# Autodesk Inventor assembly: largeCapAssemblyGlued
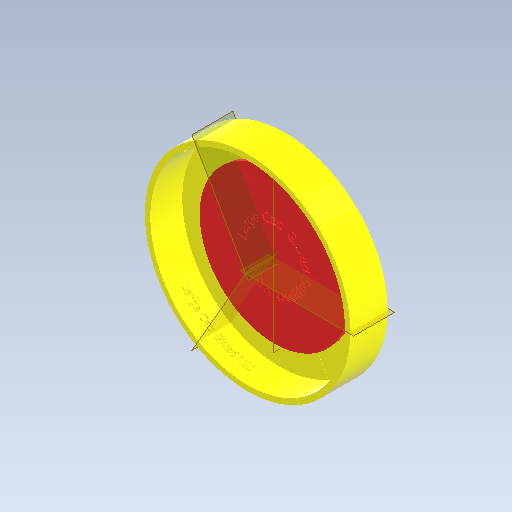
[picture p0: Inventor's stored thumbnail of the model, 512x512]
Saved by Autodesk Inventor 2021.1 (Build 251245000, 245)
## iProperties
Created: 2020-09-25
Part Number: largeCapAssemblyGlued
Document SubType Name: Assembly
Designer: robst
Author: robst
## Documents named in this file (3)
- C:\git\CAD-Development\robSteele\HouseProjects\Garage\CapForWater\largeCapAssemblyGlued.iam
- C:\git\CAD-Development\robSteele\HouseProjects\Garage\CapForWater\supportForLargeCap.ipt
- C:\git\CAD-Development\robSteele\HouseProjects\Garage\CapForWater\largeCap.ipt
## Components (4 placed, 2 different names)
1. supportForLargeCap:1 — Flush:1, Mate:1, Mate:2
2. largeCap:1 — Flush:1, Mate:1, Mate:2
3. largeCap:2
4. largeCap:3
## Component patterns: (3 elements, first: largeCap:1)
## Relationships (3: Mate 2, Flush 1)
- Flush:1: supportForLargeCap:1 ↔ largeCap:1
- Mate:1: supportForLargeCap:1 ↔ largeCap:1
- Mate:2: supportForLargeCap:1 ↔ largeCap:1
